# Autodesk Inventor assembly: 000 ASY GBK Gubkinskiy
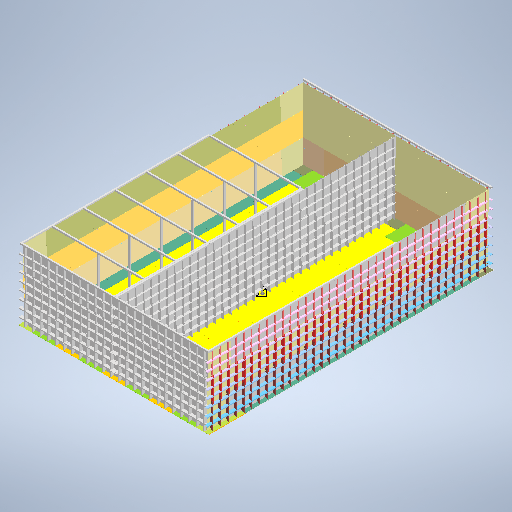
[picture p0: Inventor's stored thumbnail of the model, 512x512]
Saved by Autodesk Inventor 2026 (Build 300175000, 175)
## iProperties
Created: 2026-04-17
Part Number: 000 ASY GBK Gubkinskiy
Document SubType Name: Assembly
Designer: admin
Mass: 2.0116e+07 g
Surface Area: 1.3016e+07 cm^2
Volume: 2.56254e+06 cm^3
Density: 7.85 g/cm^3
Author: admin
## Documents named in this file (6)
- C:\Users\user\Documents\Inventor\GBK-Gubkinskiy\000 ASY GBK Gubkinskiy.iam
- C:\Users\user\Documents\Inventor\GBK-Gubkinskiy\ASY GBK длинная стенка.iam
- C:\Users\user\Documents\Inventor\GBK-Gubkinskiy\090 ASY bottom.iam
- C:\Users\user\Documents\Inventor\GBK-Gubkinskiy\ASY GBK короткая стенка.iam
- C:\Users\user\Documents\Inventor\GBK-Gubkinskiy\ASY GBK центральная стенка.iam
- C:\Users\user\Documents\Inventor\GBK-Gubkinskiy\010 ASY GBK Tube frame 1.iam
## Components (7 placed, 5 different names)
1. ASY GBK длинная стенка:1 [sub-assembly]
2. ASY GBK длинная стенка:2 [sub-assembly]
3. 090 ASY bottom:1 [sub-assembly] — Заподлицо:26, Совмещение:28, Заподлицо:27
4. ASY GBK короткая стенка:1 [sub-assembly] — Совмещение:27
5. ASY GBK короткая стенка:2 [sub-assembly]
6. ASY GBK центральная стенка:1 [sub-assembly] — Заподлицо:18, Совмещение:27
7. 010 ASY GBK Tube frame 1:1 [sub-assembly] — Заподлицо:23, Заподлицо:24, Заподлицо:25
## Relationships (8: Flush 6, Mate 2)
- Заподлицо:18 [Flush] (-2 mm): ASY GBK центральная стенка:1
- Совмещение:27 [Mate] (1.254 mm): ASY GBK короткая стенка:1 ↔ ASY GBK центральная стенка:1
- Заподлицо:23 [Flush]: 010 ASY GBK Tube frame 1:1
- Заподлицо:24 [Flush]: 010 ASY GBK Tube frame 1:1
- Заподлицо:25 [Flush]: 010 ASY GBK Tube frame 1:1
- Заподлицо:26 [Flush]: 090 ASY bottom:1
- Совмещение:28 [Mate]: 090 ASY bottom:1
- Заподлицо:27 [Flush]: 090 ASY bottom:1
## Named parameters: Зазор_по_горизонту = 1 mm, d120_Зазор_по_горизонту = 1 mm, d141_Зазор_по_горизонту = 1 mm, d159_d141_Зазор_по_горизонту = 1 mm, d175_d141_Зазор_по_горизонту = 1 mm
